# Autodesk Inventor assembly: Filament Path Assembly
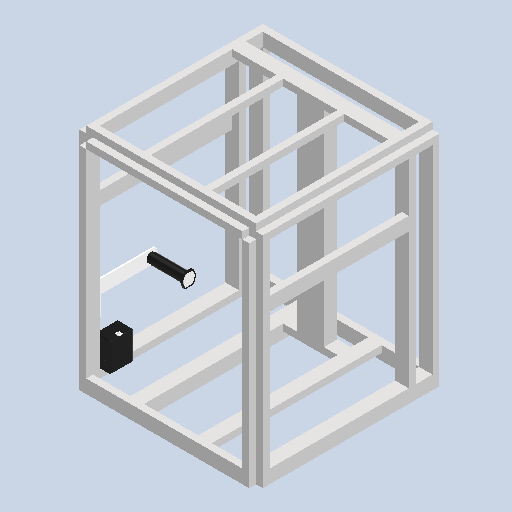
[picture p0: Inventor's stored thumbnail of the model, 512x512]
Saved by Autodesk Inventor 2024 (Build 280153000, 153)
## iProperties
Created: 2025-01-02
Part Number: Filament Path Assembly
Document SubType Name: Assembly
Designer: Ishaan
Author: Ishaan
## Documents named in this file (5)
- E:\Projects\Axiom--IDEX-3D-Printer\CAD\06 - Filament Path\Filament Path Assembly.iam
- E:\Projects\Axiom--IDEX-3D-Printer\CAD\Rev V Envelope Frame Study.ipt
- E:\Projects\Axiom--IDEX-3D-Printer\CAD\06 - Filament Path\Spool Holder Left.ipt
- E:\Projects\Axiom--IDEX-3D-Printer\CAD\06 - Filament Path\Spool Stud.ipt
- E:\Projects\Axiom--IDEX-3D-Printer\CAD\06 - Filament Path\Filament Lift Extruder.iam
## Components (4 placed, 4 different names)
1. Rev V Envelope Frame Study:1 — Mate:1, Flush:1, Mate:2, Mate:3, Mate:4, Mate:5
2. Spool Holder Left:1 — Mate:1, Flush:1, Insert:1, Insert:2
3. Spool Stud:1 — Insert:1, Insert:2, Mate:2
4. Filament Lift Extruder:1 [sub-assembly] — Mate:3, Mate:4, Mate:5
## Relationships (8: Mate 5, Insert 2, Flush 1)
- Mate:1: Rev V Envelope Frame Study:1 ↔ Spool Holder Left:1
- Flush:1 (-1 mm): Rev V Envelope Frame Study:1 ↔ Spool Holder Left:1
- Insert:1: Spool Holder Left:1 ↔ Spool Stud:1
- Insert:2: Spool Holder Left:1 ↔ Spool Stud:1
- Mate:2 (180 mm): Rev V Envelope Frame Study:1 ↔ Spool Stud:1
- Mate:3 (-17 mm): Rev V Envelope Frame Study:1 ↔ Filament Lift Extruder:1
- Mate:4 (3 mm): Rev V Envelope Frame Study:1 ↔ Filament Lift Extruder:1
- Mate:5 (3 mm): Rev V Envelope Frame Study:1 ↔ Filament Lift Extruder:1
